# Autodesk Inventor assembly: BoltAssembly
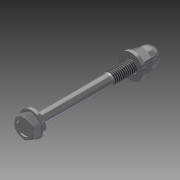
[picture p0: Inventor's stored thumbnail of the model, 180x180]
Saved by Autodesk Inventor 2015 SP1 (Build 190203100, 203)
## iProperties
Created: 2014-08-08
Part Number: BoltAssembly
Document SubType Name: Assembly
Designer: Patrick Camilleri
Author: Patrick Camilleri
## Documents named in this file (4)
- C:\Users\Patrick\CAD\Spin5 Enclosure\BoltAssembly.iam
- C:\Users\Patrick\Documents\Inventor\Content Center Files\R2015\en-US\DIN EN ISO 4015\DIN EN ISO 4015 - M6x60 x DIN EN ISO 4015.ipt
- C:\Users\Patrick\Documents\Inventor\Content Center Files\R2015\en-US\ANSI B18.22 M\ANSI B18.22M - 6 N.ipt
- C:\Users\Patrick\Documents\Inventor\Content Center Files\R2015\en-US\DIN 1587\DIN 1587 - M6 x 1.ipt
## Components (4 placed, 3 different names)
1. DIN EN ISO 4015 M6x60:1 — Mate:1, Mate:3
2. Plain Washer (Metric) 6 N:2 — Mate:2
3. Plain Washer (Metric) 6 N:1 — Mate:1, Mate:2, Mate:4
4. DIN 1587 M6:1 — Mate:3, Mate:4
## Relationships (5: Mate 4, WeldJoint 1)
- [WeldJoint]: DIN EN ISO 4015 M6x60:1 ↔ Plain Washer (Metric) 6 N:2
- Mate:1: DIN EN ISO 4015 M6x60:1 ↔ Plain Washer (Metric) 6 N:1
- Mate:2 (52 mm): Plain Washer (Metric) 6 N:2 ↔ Plain Washer (Metric) 6 N:1
- Mate:3: DIN EN ISO 4015 M6x60:1 ↔ DIN 1587 M6:1
- Mate:4: Plain Washer (Metric) 6 N:1 ↔ DIN 1587 M6:1
